# Autodesk Inventor assembly: Chair Complete
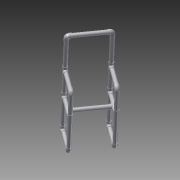
[picture p0: Inventor's stored thumbnail of the model, 180x180]
Saved by Autodesk Inventor 2015 (Build 190159000, 159)
## iProperties
Created: 2015-05-04
Part Number: Chair Complete
Document SubType Name: Assembly
Designer: 1750019
Author: 1750019
## Documents named in this file (5)
- R:\VD Proj\Chair Complete.iam
- R:\VD Proj\Chair-Side.iam
- R:\VD Proj\18 in Seg.ipt
- R:\VD Proj\MCMasterCarr\Imported Components\TEE - 4880K460\TEE - 4880K460.ipt
- R:\VD Proj\Chair-Side-Mir.iam
## Components (6 placed, 4 different names)
1. Chair-Side:1 [sub-assembly] — Rigid:3, Cylindrical:1, Mate:1
2. 18 in Seg:2 — Rigid:3, Rigid:4
3. Chair-Side-Mir:1 [sub-assembly] — Rigid:4, Cylindrical:2, Mate:2, Angle:1
4. 18 in Seg:3 — Cylindrical:3, Rigid:5, Angle:1
5. TEE - 4880K460:1 — Cylindrical:1, Mate:1, Cylindrical:4, Rigid:5
6. TEE - 4880K460:2 — Cylindrical:2, Mate:2, Cylindrical:3, Cylindrical:4
## Relationships (10: CylindricalJoint 4, WeldJoint 3, Mate 2, Angle 1)
- Rigid:3 [WeldJoint]: Chair-Side:1 ↔ 18 in Seg:2
- Rigid:4 [WeldJoint]: 18 in Seg:2 ↔ Chair-Side-Mir:1
- Cylindrical:1: Chair-Side:1 ↔ TEE - 4880K460:1
- Cylindrical:2: Chair-Side-Mir:1 ↔ TEE - 4880K460:2
- Mate:1: Chair-Side:1 ↔ TEE - 4880K460:1
- Mate:2: Chair-Side-Mir:1 ↔ TEE - 4880K460:2
- Cylindrical:3: 18 in Seg:3 ↔ TEE - 4880K460:2
- Cylindrical:4: TEE - 4880K460:1 ↔ TEE - 4880K460:2
- Rigid:5 [WeldJoint]: 18 in Seg:3 ↔ TEE - 4880K460:1
- Angle:1 (90 deg): Chair-Side-Mir:1 ↔ 18 in Seg:3
